# Autodesk Inventor assembly: КВ33.044.300 -  Сборка мотора Makeblock с крепление
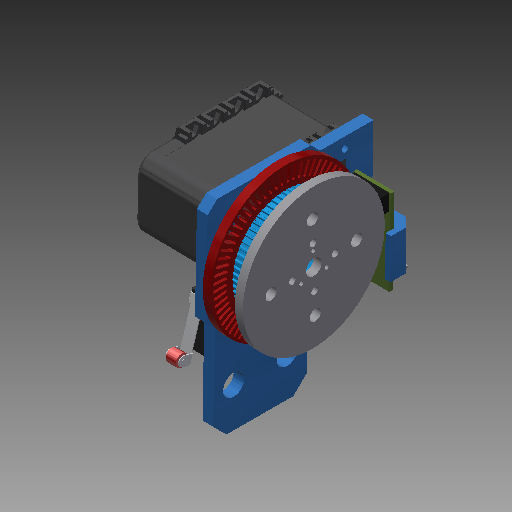
[picture p0: Inventor's stored thumbnail of the model, 512x512]
Saved by Autodesk Inventor 2019 (Build 230136000, 136)
## iProperties
Created: 2019-07-17
Part Number: КВ33.044.300 -  Сборка мотора Makeblock с крепление
Material: Типовые
Document SubType Name: Assembly
Designer: Петров Иван
Author: Петров Иван
## Documents named in this file (9)
- E:\IVAN\Kvantoriada2019\optimal_gripper\hardware\КВ33.044.400 -  Сборка сервомотора Dynamixel с крепление.iam
- E:\IVAN\Kvantoriada2019\optimal_gripper\hardware\КВ33.044.401 - Деражатель мотора.ipt
- E:\IVAN\Kvantoriada2019\optimal_gripper\hardware\КВ33.044.404 -Проставка 4.ipt
- E:\IVAN\Kvantoriada2019\optimal_gripper\hardware\КВ33.044.404 - Колесо энкодера.ipt
- E:\IVAN\Kvantoriada2019\optimal_gripper\hardware\Стандартные изделия\Шкив большой Makeblock.ipt
- E:\IVAN\Kvantoriada2019\optimal_gripper\hardware\Стандартные изделия\Сервомотор Dynamixel AX-12A\ax-12a.iam
- E:\IVAN\Kvantoriada2019\optimal_gripper\hardware\КВ33.044.405 -  Боковина шкива.ipt
- E:\IVAN\Kvantoriada2019\optimal_gripper\hardware\Стандартные изделия\Датчик оптический (с контактами с противоположной стороны).ipt
- E:\IVAN\Kvantoriada2019\optimal_gripper\hardware\Стандартные изделия\Концевик механический\Концевик механический.ipt
## Components (8 placed, 8 different names)
1. КВ33.044.401 - Деражатель мотора:1 — Совмещение:1, Совмещение:2, Совмещение:7, Совмещение:8, Совмещение:9, Заподлицо:1, Совмещение:19, Заподлицо:2, Совмещение:20, Совмещение:21, Совмещение:22
2. КВ33.044.404 -Проставка 4:1 — Совмещение:1, Совмещение:2, Совмещение:10, Совмещение:11, Совмещение:12
3. Шкив большой Makeblock:1 — Совмещение:13, Совмещение:14, Совмещение:15, Совмещение:16, Совмещение:17, Совмещение:18
4. ax-12a:1 [sub-assembly] — Совмещение:7, Совмещение:8, Совмещение:9
5. КВ33.044.404 - Колесо энкодера:1 — Совмещение:10, Совмещение:11, Совмещение:12, Совмещение:13, Совмещение:14, Совмещение:15
6. КВ33.044.405 -  Боковина шкива:1 — Совмещение:16, Совмещение:17, Совмещение:18
7. Датчик оптический (с контактами с противоположной стороны):1 — Заподлицо:1, Совмещение:19, Заподлицо:2
8. Концевик механический:1 — Совмещение:20, Совмещение:21, Совмещение:22
## Relationships (20: Mate 18, Flush 2)
- Совмещение:1 [Mate]: КВ33.044.401 - Деражатель мотора:1 ↔ КВ33.044.404 -Проставка 4:1
- Совмещение:2 [Mate]: КВ33.044.401 - Деражатель мотора:1 ↔ КВ33.044.404 -Проставка 4:1
- Совмещение:7 [Mate]: КВ33.044.401 - Деражатель мотора:1 ↔ ax-12a:1
- Совмещение:8 [Mate]: КВ33.044.401 - Деражатель мотора:1 ↔ ax-12a:1
- Совмещение:9 [Mate]: КВ33.044.401 - Деражатель мотора:1 ↔ ax-12a:1
- Совмещение:10 [Mate]: КВ33.044.404 -Проставка 4:1 ↔ КВ33.044.404 - Колесо энкодера:1
- Совмещение:11 [Mate]: КВ33.044.404 -Проставка 4:1 ↔ КВ33.044.404 - Колесо энкодера:1
- Совмещение:12 [Mate]: КВ33.044.404 -Проставка 4:1 ↔ КВ33.044.404 - Колесо энкодера:1
- Совмещение:13 [Mate]: Шкив большой Makeblock:1 ↔ КВ33.044.404 - Колесо энкодера:1
- Совмещение:14 [Mate]: Шкив большой Makeblock:1 ↔ КВ33.044.404 - Колесо энкодера:1
- Совмещение:15 [Mate]: Шкив большой Makeblock:1 ↔ КВ33.044.404 - Колесо энкодера:1
- Совмещение:16 [Mate]: Шкив большой Makeblock:1 ↔ КВ33.044.405 -  Боковина шкива:1
- Совмещение:17 [Mate]: Шкив большой Makeblock:1 ↔ КВ33.044.405 -  Боковина шкива:1
- Совмещение:18 [Mate]: Шкив большой Makeblock:1 ↔ КВ33.044.405 -  Боковина шкива:1
- Заподлицо:1 [Flush] (6 mm): КВ33.044.401 - Деражатель мотора:1 ↔ Датчик оптический (с контактами с противоположной стороны):1
- Совмещение:19 [Mate]: КВ33.044.401 - Деражатель мотора:1 ↔ Датчик оптический (с контактами с противоположной стороны):1
- Заподлицо:2 [Flush] (13 mm): КВ33.044.401 - Деражатель мотора:1 ↔ Датчик оптический (с контактами с противоположной стороны):1
- Совмещение:20 [Mate]: КВ33.044.401 - Деражатель мотора:1 ↔ Концевик механический:1
- Совмещение:21 [Mate]: КВ33.044.401 - Деражатель мотора:1 ↔ Концевик механический:1
- Совмещение:22 [Mate]: КВ33.044.401 - Деражатель мотора:1 ↔ Концевик механический:1
